# Autodesk Inventor assembly: Lift_V2
(part 2 of 2)
- Mate:141: Wall_Front:1 ↔ ISO 4032 M3:24
- Mate:142: Wall:1 ↔ ISO 4032 M3:24
- Angle:2 (0 deg): Wall:1 ↔ ISO 4032 M3:24
- Angle:3 (0 deg): Wall_Front:1 ↔ ISO 4032 M3:23
- Angle:4 (0 deg): Wall:1 ↔ ISO 4032 M3:22
- Angle:5 (0 deg): Wall_Front:1 ↔ ISO 4032 M3:21
- Angle:6 (0 deg): Wall:1 ↔ ISO 4032 M3:20
- Angle:7 (0 deg): Wall_Front:1 ↔ ISO 4032 M3:19
- Angle:8 (0 deg): Wall_Left:1 ↔ ISO 4032 M3:18
- Angle:9 (0 deg): Wall_Front:1 ↔ ISO 4032 M3:17
- Angle:10 (0 deg): Wall_Left:1 ↔ ISO 4032 M3:16
- Angle:11 (0 deg): Wall_Front:1 ↔ ISO 4032 M3:15
- Angle:12 (0 deg): Wall_Left:1 ↔ ISO 4032 M3:14
- Angle:13 (0 deg): Wall_Front:1 ↔ ISO 4032 M3:13
- Angle:14 (0 deg): Wall_Left:1 ↔ ISO 4032 M3:12
- Angle:16 (0 deg): Wall_Left:1 ↔ ISO 4032 M3:10
- Angle:18 (0 deg): Wall_Left:1 ↔ ISO 4032 M3:8
- Angle:20 (0 deg): Wall:1 ↔ ISO 4032 M3:6
- Angle:21 (0 deg): Wall_rear:1 ↔ ISO 4032 M3:1
- Angle:22 (0 deg): Wall_rear:1 ↔ ISO 4032 M3:3
- Angle:23 (0 deg): Wall:1 ↔ ISO 4032 M3:4
- Angle:24 (0 deg): Wall_rear:1 ↔ ISO 4032 M3:5
- Mate:143: Wall:1 ↔ ISO 1207 M3 x 12:25
- Mate:144: Wall:1 ↔ ISO 1207 M3 x 12:25
- Mate:145: Wall:1 ↔ ISO 1207 M3 x 12:26
- Mate:146: Wall:1 ↔ ISO 1207 M3 x 12:26
- Mate:147: Wall:1 ↔ ISO 4032 M3:25
- Mate:148: Floor:1 ↔ ISO 4032 M3:25
- Mate:149: Wall:1 ↔ ISO 4032 M3:26
- Mate:150: Floor:1 ↔ ISO 4032 M3:26
- Angle:25 (0 deg): Floor:1 ↔ ISO 4032 M3:26
- Angle:26 (0 deg): Floor:1 ↔ ISO 4032 M3:25
- Mate:151: Wall_rear:1 ↔ Floor_Bottom:1
- Mate:152: Wall_rear:1 ↔ Floor_Bottom:1
- Mate:153: Wall_rear:1 ↔ Floor_Bottom:1
- Mate:154: Baseplate:1 ↔ ISO 1207 M3 x 16:1
- Mate:155: Baseplate:1 ↔ ISO 1207 M3 x 16:1
- Mate:156: Baseplate:1 ↔ ISO 4032 M3:27
- Mate:157: Wall:1 ↔ ISO 4032 M3:27
- Mate:158: Baseplate:1 ↔ ISO 1207 M3 x 16:2
- Mate:159: Baseplate:1 ↔ ISO 1207 M3 x 16:2
- Mate:160: Baseplate:1 ↔ ISO 4032 M3:28
- Mate:161: Wall:1 ↔ ISO 4032 M3:28
- Mate:170: Baseplate:1 ↔ ISO 1207 M3 x 16:5
- Mate:171: Baseplate:1 ↔ ISO 1207 M3 x 16:5
- Mate:172: Baseplate:1 ↔ ISO 4032 M3:31
- Mate:173: Wall_Left:1 ↔ ISO 4032 M3:31
- Mate:174: Baseplate:1 ↔ ISO 1207 M3 x 16:6
- Mate:175: Baseplate:1 ↔ ISO 1207 M3 x 16:6
- Mate:176: Baseplate:1 ↔ ISO 4032 M3:32
- Mate:177: Wall_Left:1 ↔ ISO 4032 M3:32
- [Mate] (19.5 mm): Wall_Front:1 ↔ Car_ASM:1
- [Mate] (5 mm): Wall_Left:1 ↔ Car_ASM:1
- Mate:359: Wall_Front:1 ↔ Floor_Top:1
- Mate:360: Wall_Left:1 ↔ Floor_Top:1
- Mate:361: Wall_Left:1 ↔ Floor_Top:1
- Flush:9: Floor:1 ↔ Guide Rod:1
- Mate:362: Floor:1 ↔ Guide Rod:3
- Mate:363: Floor:1 ↔ Guide Rod:2
- Mate:364: Floor_Bottom:1 ↔ Guide Rod:2
- Mate:365: Floor_Bottom:1 ↔ Guide Rod:3
- Mate:366: Floor_Bottom:1 ↔ Motor24V:1
- Mate:367: Car_ASM:1 ↔ Motor24V:1
- Mate:368: SpindleAdaptor_A:1 ↔ SpindleAdaptor_B:1
- Mate:369: SpindleAdaptor_A:1 ↔ SpindleAdaptor_B:1
- Angle:27 (180 deg): Motor24V:1 ↔ SpindleAdaptor_A:1
- Mate:371: Motor24V:1 ↔ SpindleAdaptor_A:1
- Mate:372: SpindleAdaptor_A:1 ↔ Spindle_Rod:1
- Mate:373: SpindleAdaptor_A:1 ↔ Spindle_Rod:1
- Mate:374: SpindleAdaptor_B:1 ↔ Spindle_Rod:1
- Mate:375: SpindleAdaptor_A:1 ↔ ISO 7089 3:1
- Mate:376: SpindleAdaptor_A:1 ↔ ISO 7089 3:1
- Insert:18: ISO 7089 3:1 ↔ ISO 1207 M3 x 25:1
- Mate:377: SpindleAdaptor_A:1 ↔ ISO 7089 3:2
- Mate:378: SpindleAdaptor_B:1 ↔ ISO 7089 3:2
- Insert:19: ISO 7089 3:2 ↔ ISO 4032 M3:33
- Mate:379: SpindleAdaptor_A:1 ↔ ISO 7089 3:3
- Mate:380: SpindleAdaptor_A:1 ↔ ISO 7089 3:3
- Insert:20: ISO 7089 3:3 ↔ ISO 1207 M3 x 25:2
- Mate:381: SpindleAdaptor_A:1 ↔ ISO 7089 3:4
- Mate:382: SpindleAdaptor_B:1 ↔ ISO 7089 3:4
- Insert:21: ISO 7089 3:4 ↔ ISO 4032 M3:34
- Mate:383: SpindleAdaptor_A:1 ↔ ISO 7089 3:5
- Mate:384: SpindleAdaptor_A:1 ↔ ISO 7089 3:5
- Insert:22: ISO 7089 3:5 ↔ ISO 1207 M3 x 25:3
- Mate:385: SpindleAdaptor_A:1 ↔ ISO 7089 3:6
- Mate:386: SpindleAdaptor_B:1 ↔ ISO 7089 3:6
- Insert:23: ISO 7089 3:6 ↔ ISO 4032 M3:35
- Mate:387: SpindleAdaptor_A:1 ↔ ISO 7089 3:7
- Mate:388: SpindleAdaptor_A:1 ↔ ISO 7089 3:7
- Insert:24: ISO 7089 3:7 ↔ ISO 1207 M3 x 25:4
- Mate:389: SpindleAdaptor_A:1 ↔ ISO 7089 3:8
- Mate:390: SpindleAdaptor_B:1 ↔ ISO 7089 3:8
- Insert:25: ISO 7089 3:8 ↔ ISO 4032 M3:36
- Flush:10: Wall_rear:1 ↔ Cableduct_Cover:1
- Mate:392: Cableduct_Cover:1 ↔ Cableduct_Side:1
- Flush:11: Wall_Left:1 ↔ Cover:1
- Flush:12: Cover:1 ↔ Pannel_Side:1
- Mate:393: Cover:1 ↔ Pannel_Side:2
- Mate:394: Cover:1 ↔ Pannel_Side:2
- Mate:395: Cover:1 ↔ Pannel_Side:2
- Flush:13: Pannel_Side:1 ↔ Panel:1
- Mate:396: Floor_Bottom:1 ↔ Reed_Rail:1
- Mate:397: Floor_Bottom:1 ↔ SwitchHolder_Bottom:1
- Mate:398: Floor_Bottom:1 ↔ SwitchHolder_Bottom:2
- Mate:399: Floor_Top:1 ↔ SwitchHolder_Top:1
- Mate:400: Floor_Top:1 ↔ SwitchHolder_Top:2
- Mate:401: SwitchHolder_Top:1 ↔ SwitchHolder_Top:2
- Mate:402: SwitchHolder_Bottom:1 ↔ SwitchHolder_Bottom:2
- Mate:405: SwitchHolder_Bottom:1 ↔ LimitSwitch_Big:1
- Mate:406: SwitchHolder_Bottom:1 ↔ LimitSwitch_Big:1
- Mate:407: SwitchHolder_Bottom:2 ↔ LimitSwitch_Big:1
- Mate:408: SwitchHolder_Bottom:1 ↔ LimitSwitch_Big:1
- Mate:409: Car_ASM:1 ↔ LimitSwitch_Big:1
- Mate:410 (15 mm): Wall_Left:1 ↔ SwitchHolder_Bottom:2
- Flush:14 (40 mm): Floor_Bottom:1 ↔ SwitchHolder_Bottom:1
- Mate:411: SwitchHolder_Top:2 ↔ LimitSwitch_Big:2
- Mate:412: SwitchHolder_Top:2 ↔ LimitSwitch_Big:2
- Mate:413: SwitchHolder_Top:1 ↔ LimitSwitch_Big:2
- Mate:414: SwitchHolder_Top:2 ↔ LimitSwitch_Big:2
- Flush:15: SwitchHolder_Top:2 ↔ SwitchHolder_Bottom:2
- Flush:16: SwitchHolder_Top:2 ↔ SwitchHolder_Bottom:2
- Mate:415: Car_ASM:1 ↔ LimitSwitch_Big:2
- Flush:17: Wall_Front:1 ↔ Protector_80x80:1
- Mate:416: Wall_Front:1 ↔ Protector_80x80:2
- Mate:417: Wall_Front:1 ↔ Protector_80x80:2
- Mate:418: Wall_Front:1 ↔ Protector_80x80:2
- Mate:420: Panel:1 ↔ Button_Yellow:2
- Mate:421: Panel:1 ↔ Button_Yellow:3
- Mate:422: Panel:1 ↔ Button_Yellow:1
- Mate:423: Panel:1 ↔ Button_Green:1
- Mate:424: Panel:1 ↔ Button_Red:2
- Mate:425: Panel:1 ↔ LED5mm:1
- Mate:426: Panel:1 ↔ LED5mm:1
- Mate:427: Panel:1 ↔ Button_Yellow:2
- Mate:428: Panel:1 ↔ Button_Yellow:1
- Mate:429: Panel:1 ↔ Button_Green:1
- Mate:430: Panel:1 ↔ Button_Yellow:3
- Mate:431: Panel:1 ↔ Button_Red:2
- Mate:432: Pannel_Side:2 ↔ Panel:1
- Mate:433: Pannel_Side:2 ↔ Panel:1
- Mate:434: Cover:1 ↔ Pannel_Side:1
- Mate:435: Cover:1 ↔ Pannel_Side:1
- Mate:436: Floor_Bottom:1 ↔ Guide Rod:1
- Mate:437: Protector_80x80:1 ↔ ISO 7089 3:9
- Mate:438: Protector_80x80:1 ↔ ISO 7089 3:9
- Insert:26: ISO 7089 3:9 ↔ ISO 1207 M3 x 12:27
- Mate:439: Protector_80x80:1 ↔ ISO 7089 3:10
- Mate:440: Wall_Front:1 ↔ ISO 7089 3:10
- Insert:27: ISO 7089 3:10 ↔ ISO 4032 M3:37
- Mate:441: Protector_80x80:1 ↔ ISO 7089 3:11
- Mate:442: Protector_80x80:1 ↔ ISO 7089 3:11
- Insert:28: ISO 7089 3:11 ↔ ISO 1207 M3 x 12:28
- Mate:443: Protector_80x80:1 ↔ ISO 7089 3:12
- Mate:444: Wall_Front:1 ↔ ISO 7089 3:12
- Insert:29: ISO 7089 3:12 ↔ ISO 4032 M3:38
- Mate:445: Protector_80x80:1 ↔ ISO 7089 3:13
- Mate:446: Protector_80x80:1 ↔ ISO 7089 3:13
- Insert:30: ISO 7089 3:13 ↔ ISO 1207 M3 x 12:29
- Mate:447: Protector_80x80:1 ↔ ISO 7089 3:14
- Mate:448: Wall_Front:1 ↔ ISO 7089 3:14
- Insert:31: ISO 7089 3:14 ↔ ISO 4032 M3:39
- Mate:449: Protector_80x80:1 ↔ ISO 7089 3:15
- Mate:450: Protector_80x80:1 ↔ ISO 7089 3:15
- Insert:32: ISO 7089 3:15 ↔ ISO 1207 M3 x 12:30
- Mate:451: Protector_80x80:1 ↔ ISO 7089 3:16
- Mate:452: Wall_Front:1 ↔ ISO 7089 3:16
- Insert:33: ISO 7089 3:16 ↔ ISO 4032 M3:40
- Mate:453: Protector_80x80:2 ↔ ISO 7089 3:17
- Mate:454: Protector_80x80:2 ↔ ISO 7089 3:17
- Insert:34: ISO 7089 3:17 ↔ ISO 1207 M3 x 12:31
- Mate:455: Protector_80x80:2 ↔ ISO 7089 3:18
- Mate:456: Wall_Front:1 ↔ ISO 7089 3:18
- Insert:35: ISO 7089 3:18 ↔ ISO 4032 M3:41
- Mate:457: Protector_80x80:2 ↔ ISO 7089 3:19
- Mate:458: Protector_80x80:2 ↔ ISO 7089 3:19
- Insert:36: ISO 7089 3:19 ↔ ISO 1207 M3 x 12:32
- Mate:459: Protector_80x80:2 ↔ ISO 7089 3:20
- Mate:460: Wall_Front:1 ↔ ISO 7089 3:20
- Insert:37: ISO 7089 3:20 ↔ ISO 4032 M3:42
- Mate:461: Protector_80x80:2 ↔ ISO 7089 3:21
- Mate:462: Protector_80x80:2 ↔ ISO 7089 3:21
- Insert:38: ISO 7089 3:21 ↔ ISO 1207 M3 x 12:33
- Mate:463: Protector_80x80:2 ↔ ISO 7089 3:22
- Mate:464: Wall_Front:1 ↔ ISO 7089 3:22
- Insert:39: ISO 7089 3:22 ↔ ISO 4032 M3:43
- Mate:465: Protector_80x80:2 ↔ ISO 7089 3:23
- Mate:466: Protector_80x80:2 ↔ ISO 7089 3:23
- Insert:40: ISO 7089 3:23 ↔ ISO 1207 M3 x 12:34
- Mate:467: Protector_80x80:2 ↔ ISO 7089 3:24
- Mate:468: Wall_Front:1 ↔ ISO 7089 3:24
- Insert:41: ISO 7089 3:24 ↔ ISO 4032 M3:44
- Mate:469: Wall_Front:1 ↔ ISO 1207 M3 x 12:35
- Mate:470: Wall_Front:1 ↔ ISO 1207 M3 x 12:35
- Mate:471: Wall_Front:1 ↔ ISO 4032 M3:45
- Mate:472: Floor_Bottom:1 ↔ ISO 4032 M3:45
- Mate:473: Wall_Front:1 ↔ ISO 1207 M3 x 12:36
- Mate:474: Wall_Front:1 ↔ ISO 1207 M3 x 12:36
- Mate:475: Wall_Front:1 ↔ ISO 4032 M3:46
- Mate:476: Floor:1 ↔ ISO 4032 M3:46
- Mate:477: Wall_Front:1 ↔ ISO 1207 M3 x 12:37
- Mate:478: Wall_Front:1 ↔ ISO 1207 M3 x 12:37
- Mate:479: Wall_Front:1 ↔ ISO 4032 M3:47
- Mate:480: Floor_Bottom:1 ↔ ISO 4032 M3:47
- Mate:481: Wall_Front:1 ↔ ISO 1207 M3 x 12:38
- Mate:482: Wall_Front:1 ↔ ISO 1207 M3 x 12:38
- Mate:483: Wall_Front:1 ↔ ISO 4032 M3:48
- Mate:484: Floor:1 ↔ ISO 4032 M3:48
- Mate:485: Wall_Front:1 ↔ ISO 1207 M3 x 12:39
- Mate:486: Wall_Front:1 ↔ ISO 1207 M3 x 12:39
- Mate:487: Wall_Front:1 ↔ ISO 4032 M3:49
- Mate:488: Floor_Top:1 ↔ ISO 4032 M3:49
- Mate:489: Wall_Front:1 ↔ ISO 1207 M3 x 12:40
- Mate:490: Wall_Front:1 ↔ ISO 1207 M3 x 12:40
- Mate:491: Wall_Front:1 ↔ ISO 4032 M3:50
- Mate:492: Floor_Top:1 ↔ ISO 4032 M3:50
- Mate:493: Wall_rear:1 ↔ ISO 1207 M3 x 12:41
- Mate:494: Wall_rear:1 ↔ ISO 1207 M3 x 12:41
- Mate:495: Wall_rear:1 ↔ ISO 4032 M3:51
- Mate:496: Floor_Bottom:1 ↔ ISO 4032 M3:51
- Mate:497: Wall_rear:1 ↔ ISO 1207 M3 x 12:42
- Mate:498: Wall_rear:1 ↔ ISO 1207 M3 x 12:42
- Mate:499: Wall_rear:1 ↔ ISO 4032 M3:52
- Mate:500: Floor_Bottom:1 ↔ ISO 4032 M3:52
- Mate:501: Wall_rear:1 ↔ ISO 1207 M3 x 12:43
- Mate:502: Wall_rear:1 ↔ ISO 1207 M3 x 12:43
- Mate:503: Wall_rear:1 ↔ ISO 4032 M3:53
- Mate:504: Floor:1 ↔ ISO 4032 M3:53
- Mate:505: Wall_rear:1 ↔ ISO 1207 M3 x 12:44
- Mate:506: Wall_rear:1 ↔ ISO 1207 M3 x 12:44
- Mate:507: Wall_rear:1 ↔ ISO 4032 M3:54
- Mate:508: Floor:1 ↔ ISO 4032 M3:54
- Mate:509: Wall_rear:1 ↔ ISO 1207 M3 x 12:45
- Mate:510: Wall_rear:1 ↔ ISO 1207 M3 x 12:45
- Mate:511: Wall_rear:1 ↔ ISO 4032 M3:55
- Mate:512: Floor_Top:1 ↔ ISO 4032 M3:55
- Mate:513: Wall_rear:1 ↔ ISO 1207 M3 x 12:46
- Mate:514: Wall_rear:1 ↔ ISO 1207 M3 x 12:46
- Mate:515: Wall_rear:1 ↔ ISO 4032 M3:56
- Mate:516: Floor_Top:1 ↔ ISO 4032 M3:56
- Mate:517: Cover:1 ↔ ISO 1207 M3 x 12:47
- Mate:518: Cover:1 ↔ ISO 1207 M3 x 12:47
- Mate:519: Cover:1 ↔ ISO 4032 M3:57
- Mate:520: Wall_rear:1 ↔ ISO 4032 M3:57
- Mate:521: Cover:1 ↔ ISO 1207 M3 x 12:48
- Mate:522: Cover:1 ↔ ISO 1207 M3 x 12:48
- Mate:523: Cover:1 ↔ ISO 4032 M3:58
- Mate:524: Wall_rear:1 ↔ ISO 4032 M3:58
- Mate:525: Cover:1 ↔ ISO 1207 M3 x 12:49
- Mate:526: Cover:1 ↔ ISO 1207 M3 x 12:49
- Mate:527: Cover:1 ↔ ISO 4032 M3:59
- Mate:528: Wall_Left:1 ↔ ISO 4032 M3:59
- Mate:529: Cover:1 ↔ ISO 1207 M3 x 12:50
- Mate:530: Cover:1 ↔ ISO 1207 M3 x 12:50
- Mate:531: Cover:1 ↔ ISO 4032 M3:60
- Mate:532: Wall_Left:1 ↔ ISO 4032 M3:60
- Mate:533: Cover:1 ↔ ISO 1207 M3 x 12:51
- Mate:534: Cover:1 ↔ ISO 1207 M3 x 12:51
- Mate:535: Cover:1 ↔ ISO 4032 M3:61
- Mate:536: Wall_Front:1 ↔ ISO 4032 M3:61
- Mate:537: Cover:1 ↔ ISO 1207 M3 x 12:52
- Mate:538: Cover:1 ↔ ISO 1207 M3 x 12:52
- Mate:539: Cover:1 ↔ ISO 4032 M3:62
- Mate:540: Wall_Front:1 ↔ ISO 4032 M3:62
- Mate:541: Pannel_Side:2 ↔ ISO 1207 M3 x 12:53
- Mate:542: Pannel_Side:2 ↔ ISO 1207 M3 x 12:53
- Mate:543: Pannel_Side:2 ↔ ISO 4032 M3:63
- Mate:544: Panel:1 ↔ ISO 4032 M3:63
- Mate:545: Pannel_Side:2 ↔ ISO 1207 M3 x 12:54
- Mate:546: Pannel_Side:2 ↔ ISO 1207 M3 x 12:54
- Mate:547: Pannel_Side:2 ↔ ISO 4032 M3:64
- Mate:548: Panel:1 ↔ ISO 4032 M3:64
- Mate:549: Pannel_Side:1 ↔ ISO 1207 M3 x 12:55
- Mate:550: Pannel_Side:1 ↔ ISO 1207 M3 x 12:55
- Mate:551: Pannel_Side:1 ↔ ISO 4032 M3:65
- Mate:552: Panel:1 ↔ ISO 4032 M3:65
- Mate:553: Pannel_Side:1 ↔ ISO 1207 M3 x 12:56
- Mate:554: Pannel_Side:1 ↔ ISO 1207 M3 x 12:56
- Mate:555: Pannel_Side:1 ↔ ISO 4032 M3:66
- Mate:556: Panel:1 ↔ ISO 4032 M3:66
- Mate:557: Cover:1 ↔ ISO 1207 M3 x 12:57
- Mate:558: Cover:1 ↔ ISO 1207 M3 x 12:57
- Mate:559: Cover:1 ↔ ISO 4032 M3:67
- Mate:560: Pannel_Side:2 ↔ ISO 4032 M3:67
- Mate:561: Cover:1 ↔ ISO 1207 M3 x 12:58
- Mate:562: Cover:1 ↔ ISO 1207 M3 x 12:58
- Mate:563: Cover:1 ↔ ISO 4032 M3:68
- Mate:564: Pannel_Side:2 ↔ ISO 4032 M3:68
- Mate:565: Cover:1 ↔ ISO 1207 M3 x 12:59
- Mate:566: Cover:1 ↔ ISO 1207 M3 x 12:59
- Mate:567: Cover:1 ↔ ISO 4032 M3:69
- Mate:568: Pannel_Side:1 ↔ ISO 4032 M3:69
- Mate:569: Cover:1 ↔ ISO 1207 M3 x 12:60
- Mate:570: Cover:1 ↔ ISO 1207 M3 x 12:60
- Mate:571: Cover:1 ↔ ISO 4032 M3:70
- Mate:572: Pannel_Side:1 ↔ ISO 4032 M3:70
- Mate:573: Wall_rear:1 ↔ ISO 1207 M3 x 12:61
- Mate:574: Wall_rear:1 ↔ ISO 1207 M3 x 12:61
- Mate:575: Wall_rear:1 ↔ ISO 4032 M3:71
- Mate:576: Cableduct_Cover:1 ↔ ISO 4032 M3:71
- Mate:577: Cableduct_Cover:1 ↔ ISO 1207 M3 x 12:62
- Mate:578: Cableduct_Cover:1 ↔ ISO 1207 M3 x 12:62
- Mate:579: Cableduct_Cover:1 ↔ ISO 4032 M3:72
- Mate:580: Wall_rear:1 ↔ ISO 4032 M3:72
- Mate:581: Wall_rear:1 ↔ ISO 1207 M3 x 12:63
- Mate:582: Wall_rear:1 ↔ ISO 1207 M3 x 12:63
- Mate:583: Wall_rear:1 ↔ ISO 4032 M3:73
- Mate:584: Cableduct_Cover:1 ↔ ISO 4032 M3:73
- Mate:585: Cableduct_Cover:1 ↔ ISO 1207 M3 x 12:64
- Mate:586: Cableduct_Cover:1 ↔ ISO 1207 M3 x 12:64
- Mate:587: Cableduct_Cover:1 ↔ ISO 1207 M3 x 12:65
- Mate:588: Cableduct_Cover:1 ↔ ISO 1207 M3 x 12:65
- Mate:589: Cableduct_Cover:1 ↔ ISO 4032 M3:74
- Mate:590: Wall_rear:1 ↔ ISO 4032 M3:74
- Mate:591: Cableduct_Cover:1 ↔ ISO 4032 M3:75
- Mate:592: Wall_rear:1 ↔ ISO 4032 M3:75
- Mate:593: Cableduct_Cover:1 ↔ ISO 1207 M3 x 12:66
- Mate:594: Cableduct_Cover:1 ↔ ISO 1207 M3 x 12:66
- Mate:595: Cableduct_Cover:1 ↔ ISO 1207 M3 x 12:67
- Mate:596: Cableduct_Cover:1 ↔ ISO 1207 M3 x 12:67
- Mate:597: Cableduct_Cover:1 ↔ ISO 1207 M3 x 12:68
- Mate:598: Cableduct_Cover:1 ↔ ISO 1207 M3 x 12:68
- Mate:599: Cableduct_Cover:1 ↔ ISO 4032 M3:76
- Mate:600: Cableduct_Side:1 ↔ ISO 4032 M3:76
- Mate:601: Cableduct_Cover:1 ↔ ISO 4032 M3:77
- Mate:602: Cableduct_Side:1 ↔ ISO 4032 M3:77
- Mate:603: Cableduct_Cover:1 ↔ ISO 4032 M3:78
- Mate:604: Cableduct_Side:1 ↔ ISO 4032 M3:78
- Mate:605: Cableduct_Side:1 ↔ ISO 1207 M3 x 12:69
- Mate:606: Cableduct_Side:1 ↔ ISO 1207 M3 x 12:69
- Mate:607: Cableduct_Side:1 ↔ ISO 4032 M3:79
- Mate:608: Cableduct_Cover:1 ↔ ISO 4032 M3:79
- Mate:609: Wall_Left:1 ↔ ISO 1207 M3 x 12:70
- Mate:610: Wall_Left:1 ↔ ISO 1207 M3 x 12:70
- Mate:611: Wall_Left:1 ↔ ISO 1207 M3 x 12:71
- Mate:612: Wall_Left:1 ↔ ISO 1207 M3 x 12:71
- Mate:613: Wall_Left:1 ↔ ISO 1207 M3 x 12:72
- Mate:614: Wall_Left:1 ↔ ISO 1207 M3 x 12:72
- Mate:615: Wall_Left:1 ↔ ISO 1207 M3 x 12:73
- Mate:616: Wall_Left:1 ↔ ISO 1207 M3 x 12:73
- Mate:617: Wall_Left:1 ↔ ISO 1207 M3 x 12:74
- Mate:618: Wall_Left:1 ↔ ISO 1207 M3 x 12:74
- Mate:619: Wall_Left:1 ↔ ISO 1207 M3 x 12:75
- Mate:620: Wall_Left:1 ↔ ISO 1207 M3 x 12:75
- Mate:621: Wall_Left:1 ↔ ISO 4032 M3:80
- Mate:622: Floor:1 ↔ ISO 4032 M3:80
- Mate:623: Wall_Left:1 ↔ ISO 4032 M3:81
- Mate:624: Floor:1 ↔ ISO 4032 M3:81
- Mate:625: Wall_Left:1 ↔ ISO 4032 M3:82
- Mate:626: Floor:1 ↔ ISO 4032 M3:82
- Mate:627: Wall_Left:1 ↔ ISO 4032 M3:83
- Mate:628: Floor:1 ↔ ISO 4032 M3:83
- Mate:629: Wall_Left:1 ↔ ISO 4032 M3:84
- Mate:630: Floor:1 ↔ ISO 4032 M3:84
- Mate:631: Wall_Left:1 ↔ ISO 4032 M3:85
- Mate:632: Floor:1 ↔ ISO 4032 M3:85
- Mate:633: Wall:1 ↔ ISO 1207 M3 x 12:76
- Mate:634: Wall:1 ↔ ISO 1207 M3 x 12:76
- Mate:635: Wall:1 ↔ ISO 1207 M3 x 12:77
- Mate:636: Wall:1 ↔ ISO 1207 M3 x 12:77
- Mate:637: Wall:1 ↔ ISO 1207 M3 x 12:78
- Mate:638: Wall:1 ↔ ISO 1207 M3 x 12:78
- Mate:639: Wall:1 ↔ ISO 1207 M3 x 12:79
- Mate:640: Wall:1 ↔ ISO 1207 M3 x 12:79
- Mate:641: Wall:1 ↔ ISO 4032 M3:86
- Mate:642: Floor_Bottom:1 ↔ ISO 4032 M3:86
- Mate:643: Wall:1 ↔ ISO 4032 M3:87
- Mate:644: Floor_Bottom:1 ↔ ISO 4032 M3:87
- Mate:645: Wall:1 ↔ ISO 4032 M3:88
- Mate:646: Floor_Bottom:1 ↔ ISO 4032 M3:88
- Mate:647: Wall:1 ↔ ISO 4032 M3:89
- Mate:648: Floor_Bottom:1 ↔ ISO 4032 M3:89
- Mate:649: Cover:1 ↔ ISO 1207 M3 x 12:80
- Mate:650: Cover:1 ↔ ISO 1207 M3 x 12:80
- Mate:651: Cover:1 ↔ ISO 1207 M3 x 12:81
- Mate:652: Cover:1 ↔ ISO 1207 M3 x 12:81
- Mate:653: Cover:1 ↔ ISO 4032 M3:90
- Mate:654: Wall:1 ↔ ISO 4032 M3:90
- Mate:655: Cover:1 ↔ ISO 4032 M3:91
- Mate:656: Wall:1 ↔ ISO 4032 M3:91
- Mate:657: Baseplate:1 ↔ ISO 1207 M3 x 16:7
- Mate:658: Baseplate:1 ↔ ISO 1207 M3 x 16:7
- Mate:659: Baseplate:1 ↔ ISO 1207 M3 x 16:8
- Mate:660: Baseplate:1 ↔ ISO 1207 M3 x 16:8
- Mate:661: Baseplate:1 ↔ ISO 4032 M3:92
- Mate:662: Wall_Front:1 ↔ ISO 4032 M3:92
- Mate:663: Baseplate:1 ↔ ISO 4032 M3:93
- Mate:664: Wall_Front:1 ↔ ISO 4032 M3:93
- Mate:665: FloorButtonHolder_Bottom_B:1 ↔ FloorButtonHolder_Front:1
- Mate:666: FloorButtonHolder_Bottom_B:1 ↔ FloorButtonHolder_Front:1
- Mate:667: FloorButtonHolder_Bottom_B:1 ↔ FloorButtonHolder_Front:1
- Mate:668: FloorButtonHolder_Bottom_B:1 ↔ FloorButtonHolder_Side:1
- Mate:669: FloorButtonHolder_Bottom_B:1 ↔ FloorButtonHolder_Side:1
- Mate:670: FloorButtonHolder_Bottom_B:1 ↔ FloorButtonHolder_Side:1
- Mate:671: FloorButtonHolder_Side:1 ↔ FloorButtonHolder_Top_A:1
- Mate:672: FloorButtonHolder_Front:1 ↔ FloorButtonHolder_Top_A:1
- Mate:673: FloorButtonHolder_Front:1 ↔ FloorButtonHolder_Top_A:1
- Mate:674: FloorButtonHolder_Back:1 ↔ FloorButtonHolder_Top_A:1
- Mate:675: FloorButtonHolder_Back:1 ↔ FloorButtonHolder_Bottom_B:1
- Mate:676: FloorButtonHolder_Back:1 ↔ FloorButtonHolder_Bottom_B:1
- Mate:677: FloorButtonHolder_Bottom_B:1 ↔ LightGate_Plate:1
- Flush:18: FloorButtonHolder_Bottom_B:1 ↔ LightGate_Plate:1
- Mate:678: FloorButtonHolder_Bottom_B:1 ↔ LightGate_Plate:1
- Mate:679: FloorButtonHolder_Top_B:1 ↔ LightGate_Plate:1
- Mate:680: FloorButtonHolder_Top_B:1 ↔ LightGate_Plate:1
- Flush:19: FloorButtonHolder_Top_B:1 ↔ LightGate_Plate:1
- Mate:681: FloorButtonHolder_Bottom_B:1 ↔ LightGate_Door:1
- Mate:682: LightGate_Door:1 ↔ LightGate_Plate:1
- Mate:683: LightGate_Door:1 ↔ LightGate_Plate:1
- Mate:684: FloorButtonHolder_Top_B:1 ↔ FloorButtonHolder_Side:2
- Mate:685: FloorButtonHolder_Top_B:1 ↔ FloorButtonHolder_Side:2
- Mate:686: FloorButtonHolder_Top_B:1 ↔ FloorButtonHolder_Side:2
- Mate:687: FloorButtonHolder_Side:2 ↔ FloorButtonHolder_Front:2
- Mate:688: FloorButtonHolder_Top_B:1 ↔ FloorButtonHolder_Front:2
- Mate:689: FloorButtonHolder_Top_B:1 ↔ FloorButtonHolder_Front:2
- Mate:690: FloorButtonHolder_Top_B:1 ↔ FloorButtonHolder_Back:2
- Mate:691: FloorButtonHolder_Top_B:1 ↔ FloorButtonHolder_Back:2
- Flush:20: FloorButtonHolder_Side:2 ↔ FloorButtonHolder_Back:2
- Mate:692: FloorButtonHolder_Bottom_A:1 ↔ FloorButtonHolder_Front:2
- Mate:693: FloorButtonHolder_Bottom_A:1 ↔ FloorButtonHolder_Side:2
- Mate:694: FloorButtonHolder_Bottom_A:1 ↔ FloorButtonHolder_Side:2
- Mate:695: Wall_Left:1 ↔ FloorButtonHolder_Top_A:1
- Flush:21: Wall_Front:1 ↔ FloorButtonHolder_Top_A:1
- Flush:22 (20 mm): Wall_Front:1 ↔ FloorButtonHolder_Front:1
- Mate:696: FloorButtonHolder_Front:2 ↔ Button_Yellow:5
- Mate:697: FloorButtonHolder_Front:1 ↔ Button_Yellow:4
- Mate:698: FloorButtonHolder_Front:2 ↔ Button_Yellow:5
- Mate:699: FloorButtonHolder_Front:1 ↔ Button_Yellow:4
- Mate:700: LightGateCard:1 ↔ LightGate_Door:1
- Mate:701: LightGateCard:1 ↔ LightGate_Door:1
- Mate:702: Wall_Left:1 ↔ ISO 1207 M3 x 12:82
- Mate:703: Wall_Left:1 ↔ ISO 1207 M3 x 12:82
- Mate:704: Wall_Left:1 ↔ ISO 1207 M3 x 12:83
- Mate:705: Wall_Left:1 ↔ ISO 1207 M3 x 12:83
- Mate:706: Wall_Left:1 ↔ ISO 1207 M3 x 12:84
- Mate:707: Wall_Left:1 ↔ ISO 1207 M3 x 12:84
- Mate:708: Wall_Left:1 ↔ ISO 1207 M3 x 12:85
- Mate:709: Wall_Left:1 ↔ ISO 1207 M3 x 12:85
- Mate:710: Wall_Left:1 ↔ ISO 4032 M3:94
- Mate:711: FloorButtonHolder_Top_A:1 ↔ ISO 4032 M3:94
- Mate:712: Wall_Left:1 ↔ ISO 4032 M3:95
- Mate:713: FloorButtonHolder_Top_A:1 ↔ ISO 4032 M3:95
- Mate:714: Wall_Left:1 ↔ ISO 4032 M3:96
- Mate:715: FloorButtonHolder_Top_A:1 ↔ ISO 4032 M3:96
- Mate:716: Wall_Left:1 ↔ ISO 4032 M3:97
- Mate:717: FloorButtonHolder_Top_A:1 ↔ ISO 4032 M3:97
- Mate:718: FloorButtonHolder_Side:2 ↔ ISO 1207 M3 x 12:86
- Mate:719: FloorButtonHolder_Side:2 ↔ ISO 1207 M3 x 12:86
- Mate:720: FloorButtonHolder_Side:1 ↔ ISO 1207 M3 x 12:87
- Mate:721: FloorButtonHolder_Side:2 ↔ ISO 1207 M3 x 12:87
- Mate:722: FloorButtonHolder_Side:2 ↔ ISO 4032 M3:98
- Mate:723: FloorButtonHolder_Bottom_A:1 ↔ ISO 4032 M3:98
- Mate:724: FloorButtonHolder_Side:1 ↔ ISO 4032 M3:99
- Mate:725: FloorButtonHolder_Bottom_A:1 ↔ ISO 4032 M3:99
- Mate:726: FloorButtonHolder_Back:1 ↔ ISO 1207 M3 x 12:88
- Mate:727: FloorButtonHolder_Back:1 ↔ ISO 1207 M3 x 12:88
- Mate:728: FloorButtonHolder_Back:1 ↔ ISO 1207 M3 x 12:89
- Mate:729: FloorButtonHolder_Back:1 ↔ ISO 1207 M3 x 12:89
- Mate:730: FloorButtonHolder_Back:2 ↔ ISO 1207 M3 x 12:90
- Mate:731: FloorButtonHolder_Back:1 ↔ ISO 1207 M3 x 12:90
- Mate:732: FloorButtonHolder_Back:2 ↔ ISO 1207 M3 x 12:91
- Mate:733: FloorButtonHolder_Back:1 ↔ ISO 1207 M3 x 12:91
- Mate:734: FloorButtonHolder_Back:1 ↔ ISO 4032 M3:100
- Mate:735: FloorButtonHolder_Top_A:1 ↔ ISO 4032 M3:100
- Mate:736: FloorButtonHolder_Back:1 ↔ ISO 4032 M3:101
- Mate:737: FloorButtonHolder_Top_A:1 ↔ ISO 4032 M3:101
- Mate:738: FloorButtonHolder_Back:2 ↔ ISO 4032 M3:102
- Mate:739: FloorButtonHolder_Top_A:1 ↔ ISO 4032 M3:102
- Mate:740: FloorButtonHolder_Back:2 ↔ ISO 4032 M3:103
- Mate:741: FloorButtonHolder_Top_A:1 ↔ ISO 4032 M3:103
- Mate:742: FloorButtonHolder_Front:1 ↔ ISO 1207 M3 x 12:92
- Mate:743: FloorButtonHolder_Front:1 ↔ ISO 1207 M3 x 12:92
- Mate:744: FloorButtonHolder_Front:2 ↔ ISO 1207 M3 x 12:93
- Mate:745: FloorButtonHolder_Front:1 ↔ ISO 1207 M3 x 12:93
- Mate:746: FloorButtonHolder_Front:1 ↔ ISO 1207 M3 x 12:94
- Mate:747: FloorButtonHolder_Front:1 ↔ ISO 1207 M3 x 12:94
- Mate:748: FloorButtonHolder_Front:2 ↔ ISO 1207 M3 x 12:95
- Mate:749: FloorButtonHolder_Front:1 ↔ ISO 1207 M3 x 12:95
- Mate:750: FloorButtonHolder_Front:1 ↔ ISO 4032 M3:104
- Mate:751: FloorButtonHolder_Top_A:1 ↔ ISO 4032 M3:104
- Mate:752: FloorButtonHolder_Front:2 ↔ ISO 4032 M3:105
- Mate:753: FloorButtonHolder_Top_A:1 ↔ ISO 4032 M3:105
- Mate:754: FloorButtonHolder_Front:1 ↔ ISO 4032 M3:106
- Mate:755: FloorButtonHolder_Top_A:1 ↔ ISO 4032 M3:106
- Mate:756: FloorButtonHolder_Front:2 ↔ ISO 4032 M3:107
- Mate:757: FloorButtonHolder_Top_A:1 ↔ ISO 4032 M3:107
- Mate:758: FloorButtonHolder_Top_A:1 ↔ ISO 1207 M3 x 12:96
- Mate:759: FloorButtonHolder_Top_A:1 ↔ ISO 1207 M3 x 12:96
- Mate:760: FloorButtonHolder_Top_A:1 ↔ ISO 4032 M3:108
- Mate:761: FloorButtonHolder_Side:1 ↔ ISO 4032 M3:108
- Mate:762: FloorButtonHolder_Bottom_B:1 ↔ ISO 1207 M3 x 12:97
- Mate:763: FloorButtonHolder_Bottom_B:1 ↔ ISO 1207 M3 x 12:97
- Mate:764: FloorButtonHolder_Bottom_B:1 ↔ ISO 4032 M3:109
- Mate:765: FloorButtonHolder_Side:1 ↔ ISO 4032 M3:109
- Mate:766: FloorButtonHolder_Top_B:1 ↔ ISO 1207 M3 x 12:98
- Mate:767: FloorButtonHolder_Top_B:1 ↔ ISO 1207 M3 x 12:98
- Mate:768: FloorButtonHolder_Top_B:1 ↔ ISO 4032 M3:110
- Mate:769: FloorButtonHolder_Side:2 ↔ ISO 4032 M3:110
- Mate:770: FloorButtonHolder_Bottom_A:1 ↔ ISO 1207 M3 x 12:99
- Mate:771: FloorButtonHolder_Bottom_A:1 ↔ ISO 1207 M3 x 12:99
- Mate:772: FloorButtonHolder_Bottom_A:1 ↔ ISO 4032 M3:111
- Mate:773: FloorButtonHolder_Side:2 ↔ ISO 4032 M3:111
- Mate:774: Wall_rear:1 ↔ Cableduct_Cover:1
- Mate:775: Cableduct_Cover:1 ↔ Cableduct_Side:1
- Mate:776: Wall_rear:1 ↔ Cableduct_Cover:1
- Mate:777: Cableduct_Cover:1 ↔ Cableduct_Side:1
- Mate:778: Baseplate_face:1 ↔ Cableduct_Cover:1
- Mate:779: Wall_rear:1 ↔ Cover:1
- Mate:780: Wall_Left:1 ↔ Cover:1
- Mate:781: Wall_Front:1 ↔ ISO 1207 M3 x 12:27
- Mate:782: Wall_Front:1 ↔ ISO 1207 M3 x 12:29
- Mate:783: Floor_Bottom:1 ↔ Reed_Rail:1
- Mate:784: Floor_Bottom:1 ↔ Reed_Rail:1
- Mate:785: Floor_Bottom:1 ↔ Reed_Rail:1
- Mate:786: Floor_Top:1 ↔ ISO 4032 M3:81
- Flush:23: Wall_rear:1 ↔ Floor:1
- Flush:24: ISO 4032 M3:37 ↔ ISO 4032 M3:40
- Angle:28 (0 deg): ISO 4032 M3:40 ↔ ISO 4032 M3:42
- Angle:29 (0 deg): ISO 4032 M3:41 ↔ ISO 4032 M3:42
- Angle:30 (0 deg): Floor_Bottom:1 ↔ ISO 4032 M3:37
- Angle:31 (0 deg): ISO 4032 M3:40 ↔ ISO 4032 M3:42
- Angle:32 (0 deg): ISO 4032 M3:37 ↔ ISO 4032 M3:41
- Angle:33 (0 deg): ISO 4032 M3:37 ↔ ISO 4032 M3:38
- Angle:34 (0 deg): ISO 4032 M3:39 ↔ ISO 4032 M3:40
- Angle:35 (0 deg): ISO 1207 M3 x 12:33 ↔ ISO 1207 M3 x 12:34
- Angle:36 (0 deg): ISO 1207 M3 x 12:27 ↔ ISO 1207 M3 x 12:30
- Angle:37 (0 deg): ISO 1207 M3 x 12:30 ↔ ISO 1207 M3 x 12:32
- Angle:38 (0 deg): ISO 1207 M3 x 12:29 ↔ ISO 1207 M3 x 12:30
- Angle:39 (0 deg): ISO 1207 M3 x 12:28 ↔ ISO 1207 M3 x 12:29
- Angle:40 (0 deg): Baseplate_face:1 ↔ ISO 1207 M3 x 12:28
- Angle:41 (0 deg): ISO 4032 M3:33 ↔ ISO 4032 M3:36
- Angle:42 (0 deg): ISO 4032 M3:33 ↔ ISO 4032 M3:34
- Angle:43 (0 deg): ISO 4032 M3:35 ↔ ISO 4032 M3:36
- Angle:44 (0 deg): Floor_Bottom:1 ↔ ISO 4032 M3:36
- Angle:45 (0 deg): Wall:1 ↔ ISO 1207 M3 x 25:1
- Mate:787: Floor_Bottom:1 ↔ ISO 1207 M3 x 5:1
- Mate:788: Floor_Bottom:1 ↔ ISO 1207 M3 x 5:1
- Mate:789: Floor_Bottom:1 ↔ ISO 1207 M3 x 5:2
- Mate:790: Floor_Bottom:1 ↔ ISO 1207 M3 x 5:2
- Mate:791: Floor_Bottom:1 ↔ ISO 1207 M3 x 5:3
- Mate:792: Floor_Bottom:1 ↔ ISO 1207 M3 x 5:3
- Mate:793: Floor_Bottom:1 ↔ ISO 1207 M3 x 5:4
- Mate:794: Floor_Bottom:1 ↔ ISO 1207 M3 x 5:4
- Mate:795: Floor_Bottom:1 ↔ ISO 1207 M3 x 5:5
- Mate:796: Floor_Bottom:1 ↔ ISO 1207 M3 x 5:5
- Mate:797: Floor_Bottom:1 ↔ ISO 1207 M3 x 5:6
- Mate:798: Floor_Bottom:1 ↔ ISO 1207 M3 x 5:6
- Angle:46 (0 deg): ISO 1207 M3 x 25:1 ↔ ISO 1207 M3 x 25:4
- Angle:47 (0 deg): ISO 1207 M3 x 25:2 ↔ ISO 1207 M3 x 25:3
- Angle:48 (0 deg): ISO 1207 M3 x 25:3 ↔ ISO 1207 M3 x 25:4
- Angle:49 (0 deg): Floor_Bottom:1 ↔ ISO 1207 M3 x 25:3
- Mate:799: Wall:1 ↔ Wall_rear:1
- Mate:800: Wall_rear:1 ↔ CoverHolder:1
- Mate:801: Wall_rear:1 ↔ CoverHolder:1
- Mate:802: Wall_rear:1 ↔ CoverHolder:1
- Mate:803: Wall_rear:1 ↔ CoverHolder:4
- Mate:804: Wall_rear:1 ↔ CoverHolder:3
- Mate:805: Wall_rear:1 ↔ CoverHolder:2
- Mate:806: Wall_rear:1 ↔ CoverHolder:3
- Mate:807: Wall_rear:1 ↔ CoverHolder:2
- Mate:808: Wall_rear:1 ↔ CoverHolder:4
- Mate:809: Wall_rear:1 ↔ CoverHolder:4
- Mate:810: Wall_rear:1 ↔ CoverHolder:2
- Mate:811: Wall_rear:1 ↔ CoverHolder:3
- Flush:25: CoverHolder:1 ↔ Cover_Back:1
- Mate:812: CoverHolder:4 ↔ Cover_Back:1
- Mate:813: CoverHolder:4 ↔ Cover_Back:1
- Mate:814: CoverHolder:1 ↔ Cover_Back:1
- Angle:50 (0 deg): Wall:1 ↔ ISO 4032 M3:27
- Angle:51 (0 deg): Wall:1 ↔ ISO 4032 M3:28
- Angle:52 (0 deg): Wall:1 ↔ ISO 4032 M3:91
- Angle:53 (0 deg): Wall:1 ↔ ISO 4032 M3:90
- Angle:54 (0 deg): Wall_Front:1 ↔ ISO 4032 M3:93
- Angle:55 (0 deg): Wall_Front:1 ↔ ISO 4032 M3:92
- Angle:56 (0 deg): Wall_Front:1 ↔ ISO 4032 M3:61
- Angle:57 (0 deg): Wall_Front:1 ↔ ISO 4032 M3:62
- Angle:58 (0 deg): Wall_Left:1 ↔ ISO 4032 M3:60
- Angle:59 (0 deg): Wall_Left:1 ↔ ISO 4032 M3:59
- Angle:60 (0 deg): Pannel_Side:1 ↔ ISO 4032 M3:69
- Angle:61 (0 deg): Pannel_Side:1 ↔ ISO 4032 M3:70
- Angle:62 (0 deg): Cableduct_Cover:1 ↔ ISO 4032 M3:71
- Angle:63 (0 deg): Wall_rear:1 ↔ ISO 4032 M3:72
- Angle:64 (0 deg): Cableduct_Cover:1 ↔ ISO 4032 M3:79
- Angle:65 (0 deg): Wall_rear:1 ↔ ISO 4032 M3:75
- Angle:66 (0 deg): Cableduct_Cover:1 ↔ ISO 4032 M3:73
- Angle:67 (0 deg): Wall_rear:1 ↔ ISO 4032 M3:74
- Angle:68 (0 deg): FloorButtonHolder_Top_B:1 ↔ ISO 4032 M3:102
- Angle:69 (0 deg): FloorButtonHolder_Top_B:1 ↔ ISO 4032 M3:96
- Angle:70 (0 deg): FloorButtonHolder_Top_A:1 ↔ ISO 4032 M3:100
- Angle:71 (0 deg): FloorButtonHolder_Top_A:1 ↔ ISO 4032 M3:94
- Angle:72 (0 deg): FloorButtonHolder_Top_A:1 ↔ ISO 4032 M3:99
- Angle:73 (0 deg): FloorButtonHolder_Top_A:1 ↔ ISO 4032 M3:104
- Angle:74 (0 deg): FloorButtonHolder_Side:1 ↔ ISO 4032 M3:108
- Angle:75 (0 deg): FloorButtonHolder_Side:1 ↔ ISO 4032 M3:109
- Angle:76 (0 deg): FloorButtonHolder_Side:2 ↔ ISO 4032 M3:110
- Angle:77 (0 deg): FloorButtonHolder_Side:2 ↔ ISO 4032 M3:111
- Angle:78 (0 deg): FloorButtonHolder_Bottom_B:1 ↔ ISO 4032 M3:106
- Angle:79 (0 deg): FloorButtonHolder_Top_B:1 ↔ ISO 4032 M3:105
- Angle:80 (0 deg): FloorButtonHolder_Bottom_A:1 ↔ ISO 4032 M3:107
- Angle:81 (0 deg): FloorButtonHolder_Bottom_A:1 ↔ ISO 4032 M3:97
- Angle:82 (0 deg): FloorButtonHolder_Bottom_A:1 ↔ ISO 4032 M3:98
- Mate:815: Wall_rear:1 ↔ ISO 1207 M3 x 12:100
- Mate:816: Wall_rear:1 ↔ ISO 1207 M3 x 12:100
- Mate:817: Wall_rear:1 ↔ ISO 1207 M3 x 12:101
- Mate:818: Wall_rear:1 ↔ ISO 1207 M3 x 12:101
- Mate:819: Wall_rear:1 ↔ ISO 1207 M3 x 12:102
- Mate:820: Wall_rear:1 ↔ ISO 1207 M3 x 12:102
- Mate:821: Wall_rear:1 ↔ ISO 1207 M3 x 12:103
- Mate:822: Wall_rear:1 ↔ ISO 1207 M3 x 12:103
- Mate:823: Wall_rear:1 ↔ ISO 4032 M3:112
- Mate:824: CoverHolder:1 ↔ ISO 4032 M3:112
- Mate:825: Wall_rear:1 ↔ ISO 4032 M3:113
- Mate:826: CoverHolder:1 ↔ ISO 4032 M3:113
- Mate:827: Wall_rear:1 ↔ ISO 4032 M3:114
- Mate:828: CoverHolder:1 ↔ ISO 4032 M3:114
- Mate:829: Wall_rear:1 ↔ ISO 4032 M3:115
- Mate:830: CoverHolder:1 ↔ ISO 4032 M3:115
- Angle:83 (0 deg): CoverHolder:1 ↔ ISO 4032 M3:113
- Angle:84 (0 deg): CoverHolder:3 ↔ ISO 4032 M3:114
- Angle:85 (0 deg): CoverHolder:2 ↔ ISO 4032 M3:115
- Angle:86 (0 deg): Floor_Bottom:1 ↔ ISO 4032 M3:51
- Angle:87 (0 deg): Floor_Bottom:1 ↔ ISO 4032 M3:52
- Angle:88 (0 deg): Floor_Bottom:1 ↔ ISO 4032 M3:45
- Angle:89 (0 deg): Floor_Bottom:1 ↔ ISO 4032 M3:47
- Angle:90 (0 deg): Floor_Bottom:1 ↔ ISO 4032 M3:83
- Angle:91 (0 deg): Floor_Bottom:1 ↔ ISO 4032 M3:82
- Mate:831: SwitchHolder_Bottom:1 ↔ ISO 7089 3:25
- Mate:832: SwitchHolder_Bottom:1 ↔ ISO 7089 3:25
- Mate:833: SwitchHolder_Bottom:1 ↔ ISO 7089 3:27
- Mate:834: SwitchHolder_Bottom:1 ↔ ISO 7089 3:27
- Insert:42: ISO 7089 3:25 ↔ ISO 1207 M3 x 25:5
- Insert:43: ISO 7089 3:27 ↔ ISO 1207 M3 x 25:6
- Mate:835: SwitchHolder_Bottom:1 ↔ ISO 7089 3:26
- Mate:836: SwitchHolder_Bottom:2 ↔ ISO 7089 3:26
- Mate:837: SwitchHolder_Bottom:1 ↔ ISO 7089 3:28
- Mate:838: SwitchHolder_Bottom:2 ↔ ISO 7089 3:28
- Insert:44: ISO 7089 3:26 ↔ ISO 4032 M3:116
- Insert:45: ISO 7089 3:28 ↔ ISO 4032 M3:117
- Mate:839: SwitchHolder_Top:1 ↔ ISO 7089 3:29
- Mate:840: SwitchHolder_Top:1 ↔ ISO 7089 3:29
- Mate:841: SwitchHolder_Top:1 ↔ ISO 7089 3:31
- Mate:842: SwitchHolder_Top:1 ↔ ISO 7089 3:31
- Insert:46: ISO 7089 3:29 ↔ ISO 1207 M3 x 25:7
- Insert:47: ISO 7089 3:31 ↔ ISO 1207 M3 x 25:8
- Mate:843: SwitchHolder_Top:1 ↔ ISO 7089 3:30
- Mate:844: SwitchHolder_Top:2 ↔ ISO 7089 3:30
- Mate:845: SwitchHolder_Top:1 ↔ ISO 7089 3:32
- Mate:846: SwitchHolder_Top:2 ↔ ISO 7089 3:32
- Insert:48: ISO 7089 3:30 ↔ ISO 4032 M3:118
- Insert:49: ISO 7089 3:32 ↔ ISO 4032 M3:119
- Mate:847: Floor_Top:1 ↔ ISO 1207 M3 x 12:104
- Mate:848: Floor_Top:1 ↔ ISO 1207 M3 x 12:104
- Mate:849: Floor_Top:1 ↔ ISO 1207 M3 x 12:105
- Mate:850: Floor_Top:1 ↔ ISO 1207 M3 x 12:105
- Mate:851: Floor_Top:1 ↔ ISO 1207 M3 x 12:106
- Mate:852: Floor_Top:1 ↔ ISO 1207 M3 x 12:106
- Mate:853: Floor_Top:1 ↔ ISO 4032 M3:120
- Mate:854: Reed_Rail:1 ↔ ISO 4032 M3:120
- Mate:855: Floor_Top:1 ↔ ISO 4032 M3:121
- Mate:856: Reed_Rail:1 ↔ ISO 4032 M3:121
- Mate:857: Floor_Top:1 ↔ ISO 4032 M3:122
- Mate:858: Reed_Rail:1 ↔ ISO 4032 M3:122
- Mate:859: Floor_Bottom:1 ↔ ISO 1207 M3 x 12:107
- Mate:860: Floor_Bottom:1 ↔ ISO 1207 M3 x 12:107
- Mate:861: Floor_Bottom:1 ↔ ISO 1207 M3 x 12:108
- Mate:862: Floor_Bottom:1 ↔ ISO 1207 M3 x 12:108
- Mate:863: Floor_Bottom:1 ↔ ISO 4032 M3:123
- Mate:864: SwitchHolder_Bottom:1 ↔ ISO 4032 M3:123
- Mate:865: Floor_Bottom:1 ↔ ISO 4032 M3:124
- Mate:866: SwitchHolder_Bottom:1 ↔ ISO 4032 M3:124
- Angle:92 (0 deg): SwitchHolder_Bottom:1 ↔ ISO 4032 M3:123
- Angle:93 (0 deg): SwitchHolder_Bottom:2 ↔ ISO 4032 M3:124
- Angle:94 (0 deg): Cableduct_Side:1 ↔ ISO 4032 M3:77
- Flush:26: SpindleAdaptor_A:1 ↔ Spindle_Bearing_Holder:1
- Flush:27: Floor_Bottom:1 ↔ Spindle_Bearing_Holder:1
- Mate:867: SpindleAdaptor_A:1 ↔ Bearing:1
- Mate:868 (6 mm): Spindle_Bearing_Holder:1 ↔ Bearing:1
- Mate:869: Spindle_Bearing_Holder:1 ↔ Bearing:1
- Mate:872: Spindle_Bearing_Holder:1 ↔ ISO 1207 M3 x 10:1
- Mate:874: Spindle_Bearing_Holder:1 ↔ ISO 1207 M3 x 10:2
- Mate:876: Spindle_Bearing_Holder:1 ↔ ISO 1207 M3 x 10:3
- Mate:878: Spindle_Bearing_Holder:1 ↔ ISO 1207 M3 x 10:4
- Mate:880: Spindle_Bearing_Holder:1 ↔ ISO 1207 M3 x 10:5
- Mate:882: Spindle_Bearing_Holder:1 ↔ ISO 1207 M3 x 10:6
- Mate:884: Floor_Bottom:1 ↔ ISO 7089 3:33
- Mate:886: Floor_Bottom:1 ↔ ISO 7089 3:34
- Mate:888: Floor_Bottom:1 ↔ ISO 7089 3:35
- Mate:890: Floor_Bottom:1 ↔ ISO 7089 3:36
- Mate:892: Floor_Bottom:1 ↔ ISO 7089 3:37
- Mate:894: Floor_Bottom:1 ↔ ISO 7089 3:38
- Insert:50: ISO 7089 3:33 ↔ ISO 4032 M3:125
- Insert:51: ISO 7089 3:34 ↔ ISO 4032 M3:126
- Insert:52: ISO 7089 3:35 ↔ ISO 4032 M3:127
- Insert:53: ISO 7089 3:36 ↔ ISO 4032 M3:128
- Insert:54: ISO 7089 3:37 ↔ ISO 4032 M3:129
- Insert:55: ISO 7089 3:38 ↔ ISO 4032 M3:130
- Mate:895: Spindle_Bearing_Holder:1 ↔ ISO 1207 M3 x 10:2
- Mate:896: Spindle_Bearing_Holder:1 ↔ ISO 1207 M3 x 10:3
- Mate:897: Spindle_Bearing_Holder:1 ↔ ISO 1207 M3 x 10:1
- Mate:898: Spindle_Bearing_Holder:1 ↔ ISO 1207 M3 x 10:4
- Mate:899: Spindle_Bearing_Holder:1 ↔ ISO 1207 M3 x 10:6
- Mate:900: Spindle_Bearing_Holder:1 ↔ ISO 1207 M3 x 10:5
- Mate:901: Floor_Bottom:1 ↔ Spindle_Bearing_Holder:1
- Mate:902: ISO 1207 M3 x 10:1 ↔ ISO 4032 M3:125
- Mate:903: ISO 1207 M3 x 10:2 ↔ ISO 4032 M3:126
- Mate:904: ISO 1207 M3 x 10:3 ↔ ISO 4032 M3:127
- Mate:905: ISO 1207 M3 x 10:4 ↔ ISO 4032 M3:128
- Mate:906: ISO 1207 M3 x 10:6 ↔ ISO 4032 M3:130
- Mate:907: ISO 1207 M3 x 10:5 ↔ ISO 4032 M3:129
- Angle:95 (0 deg): ISO 1207 M3 x 12:107 ↔ ISO 1207 M3 x 12:108
- Angle:96 (0 deg): Floor_Bottom:1 ↔ ISO 1207 M3 x 12:108
- Angle:97 (0 deg): ISO 4032 M3:126 ↔ ISO 4032 M3:127
- Angle:98 (0 deg): ISO 4032 M3:125 ↔ ISO 4032 M3:126
- Angle:99 (0 deg): Floor_Bottom:1 ↔ ISO 4032 M3:127
- Angle:100 (0 deg): ISO 4032 M3:125 ↔ ISO 4032 M3:130
- Angle:101 (0 deg): ISO 4032 M3:128 ↔ ISO 4032 M3:130
- Angle:102 (0 deg): ISO 4032 M3:126 ↔ ISO 4032 M3:130
- Angle:103 (0 deg): ISO 4032 M3:129 ↔ ISO 4032 M3:130
